# Autodesk Inventor assembly: Bearing V2
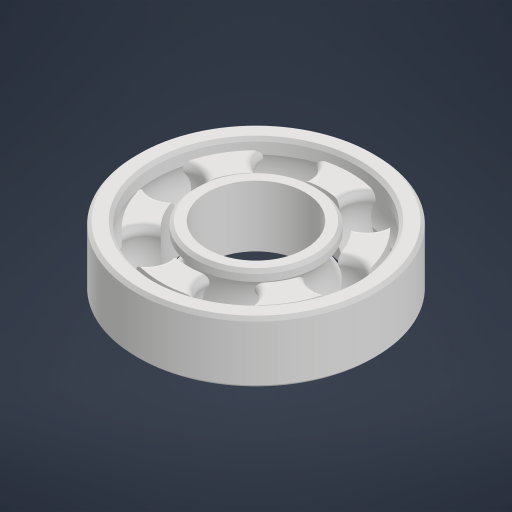
[picture p0: Inventor's stored thumbnail of the model, 512x512]
Saved by Autodesk Inventor 2023 (Build 270158000, 158)
## iProperties
Created: 2023-02-24
Part Number: Bearing V2
Document SubType Name: Assembly
Designer: izack
Author: izack
## Documents named in this file (4)
- D:\Robotics\Custom-Modules-CAD\Bearings V2\Bearing V2.iam
- D:\Robotics\Custom-Modules-CAD\Bearings V2\Parts\Inner_Ring.ipt
- D:\Robotics\Custom-Modules-CAD\Bearings V2\Outer_Ring.ipt
- D:\Robotics\Custom-Modules-CAD\Bearings V2\Parts\Spacer.ipt
## Components (3 placed, 3 different names)
1. Inner_Ring:1 — Flush:2
2. Outer_Ring:1 — Flush:1, Flush:2, Flush:3
3. Spacer:1 — Flush:3
## Relationships (3: Flush 3)
- Flush:1: Outer_Ring:1
- Flush:2: Inner_Ring:1 ↔ Outer_Ring:1
- Flush:3: Outer_Ring:1 ↔ Spacer:1
## Named parameters: di = 8 mm, p = 0 mm
